# Autodesk Inventor assembly: leg_1
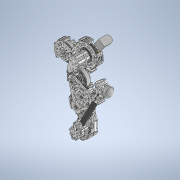
[picture p0: Inventor's stored thumbnail of the model, 180x180]
Saved by Autodesk Inventor 2020 (Build 240168000, 168)
## iProperties
Created: 2020-10-07
Part Number: leg_1
Document SubType Name: Assembly
Designer: Shuang Peng
Author: Shuang Peng
## Documents named in this file (4)
- D:\projects-3\biped_gen1\hardware\leg_1.iam
- D:\projects-3\biped_gen1\hardware\reducer_2.iam
- D:\projects-3\biped_gen1\hardware\reducer_leg.iam
- D:\projects-3\biped_gen1\hardware\sub_leg_1_lit.iam
## Components (3 placed, 3 different names)
1. reducer_2:1 [sub-assembly] — Insert:1
2. reducer_leg:1 [sub-assembly] — Insert:1, Insert:2
3. sub_leg_1_lit:1 [sub-assembly] — Insert:2
## Relationships (2: Insert 2)
- Insert:1: reducer_2:1 ↔ reducer_leg:1
- Insert:2: reducer_leg:1 ↔ sub_leg_1_lit:1
